# Autodesk Inventor assembly: RAMPSAssembled
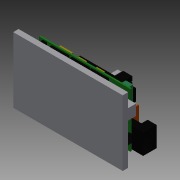
[picture p0: Inventor's stored thumbnail of the model, 180x180]
Saved by Autodesk Inventor 2015 (Build 190159000, 159)
## iProperties
Created: 2014-02-09
Part Number: RAMPSAssembled
Document SubType Name: Assembly
Designer: Jack
Author: Jack
## Documents named in this file (4)
- C:\Users\Jack\Sync\MendelMax1.5\InventorParts\Electronics\RAMPSAssembled.iam
- C:\Users\Jack\Sync\MendelMax1.5\InventorParts\Electronics\ArduinoMega.ipt
- C:\Users\Jack\Sync\MendelMax1.5\InventorParts\Electronics\RAMPS1-4.ipt
- C:\Users\Jack\Sync\MendelMax1.5\InventorParts\Electronics\RampsPly.ipt
## Components (3 placed, 3 different names)
1. ArduinoMega:1 — Mate:1, Flush:1, Mate:2, Flush:2, Flush:3
2. RAMPS1-4:1 — Mate:1, Flush:1
3. RampsPly:1 — Mate:2, Flush:2, Flush:3
## Relationships (5: Flush 3, Mate 2)
- Mate:1: ArduinoMega:1 ↔ RAMPS1-4:1
- Flush:1: ArduinoMega:1 ↔ RAMPS1-4:1
- Mate:2: ArduinoMega:1 ↔ RampsPly:1
- Flush:2 (-10 mm): ArduinoMega:1 ↔ RampsPly:1
- Flush:3 (-10 mm): ArduinoMega:1 ↔ RampsPly:1
